# Autodesk Inventor assembly: Assembled Water Sensor Chassi
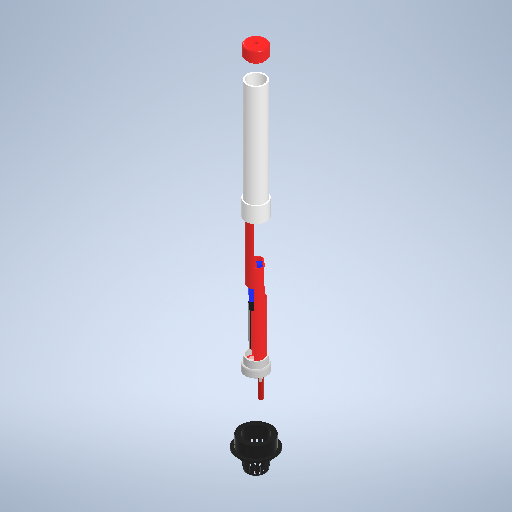
[picture p0: Inventor's stored thumbnail of the model, 512x512]
Saved by Autodesk Inventor 2025 (Build 290162000, 162)
## iProperties
Created: 2024-06-24
Part Number: Assembled Water Sensor Chassi
Document SubType Name: Assembly
Designer: track
Author: track
## Documents named in this file (14)
- C:\Users\track\OneDrive\Documents\In-Situ-Water-Quality-Sensor\System_development\Jocassee\V0.4.7\Water Sensor Chassi CAD\Assembled Water Sensor Chassi.iam
- C:\Users\track\OneDrive\Documents\In-Situ-Water-Quality-Sensor\System_development\Jocassee\V0.4.7\Water Sensor Chassi CAD\Water_Sensor_Cap.ipt
- C:\Users\track\OneDrive\Documents\In-Situ-Water-Quality-Sensor\System_development\Jocassee\V0.4.7\Tray_CAD_File\PCB tray CAD.ipt
- C:\Users\track\OneDrive\Documents\In-Situ-Water-Quality-Sensor\System_development\Jocassee\V0.4.7\Water Sensor Chassi CAD\Water Sensor Shaft (For assembly only).ipt
- C:\Users\track\OneDrive\Documents\In-Situ-Water-Quality-Sensor\System_development\Jocassee\V0.4.7\Water Sensor Chassi CAD\Male Adaptor to Water Sensor.ipt
- C:\Users\track\OneDrive\Documents\In-Situ-Water-Quality-Sensor\System_development\Jocassee\V0.4.7\Water Sensor Chassi CAD\Water Sensor Grate.ipt
- C:\Users\track\OneDrive\Documents\In-Situ-Water-Quality-Sensor\System_development\Jocassee\V0.4.7\Water Sensor Chassi CAD\Arc Water Sensor.ipt
- C:\Users\track\OneDrive\Documents\In-Situ-Water-Quality-Sensor\System_development\Jocassee\V0.4.7\Water Sensor Chassi CAD\Light Water Sensor.ipt
- C:\Users\track\OneDrive\Documents\In-Situ-Water-Quality-Sensor\System_development\Jocassee\V0.4.7\Water Sensor Chassi CAD\pH Sensor.ipt
- C:\Users\track\OneDrive\Documents\In-Situ-Water-Quality-Sensor\System_development\Jocassee\V0.4.7\Water Sensor Chassi CAD\Temp Water Sensor.ipt
- C:\Users\track\OneDrive\Documents\In-Situ-Water-Quality-Sensor\System_development\Jocassee\V0.4.7\Water Sensor Chassi CAD\PCB Board.ipt
- C:\Users\track\OneDrive\Documents\In-Situ-Water-Quality-Sensor\System_development\Jocassee\V0.4.7\Water Sensor Chassi CAD\Battery for Water Sensor.ipt
- C:\Users\track\OneDrive\Documents\In-Situ-Water-Quality-Sensor\System_development\Jocassee\V0.4.7\Tray_CAD_File\PCB Tray Top.ipt
- C:\Users\track\OneDrive\Documents\In-Situ-Water-Quality-Sensor\System_development\Jocassee\V0.4.7\Tray_CAD_File\PCB Battery Tray.ipt
## Components (13 placed, 13 different names)
1. PCB tray CAD:1 — Flush:2, Mate:2, Flush:3, Mate:3, Mate:4, Mate:5, Rigid:1, Mate:6, Mate:7, Flush:5, Mate:10, Mate:11, Mate:12, Mate:18, Mate:19, Mate:20, Mate:21, Mate:22
2. Water Sensor Shaft (For assembly only):1 — Mate:14, Mate:15
3. Water_Sensor_Cap:1 — Mate:15
4. Male Adaptor to Water Sensor:1 — Mate:11, Mate:12, Mate:13, Mate:14
5. Water Sensor Grate:1 — Mate:13
6. Arc Water Sensor:1 — Flush:5, Mate:10
7. Light Water Sensor:1 — Flush:3, Rigid:1
8. pH Sensor:1 — Mate:6, Mate:7
9. Temp Water Sensor:1 — Flush:2, Mate:2
10. PCB Board:1 — Mate:3, Mate:4, Mate:5
11. Battery for Water Sensor:1 — Mate:16, Flush:6, Mate:17
12. PCB Tray Top:1 — Mate:21, Mate:22
13. PCB Battery Tray:1 — Mate:16, Flush:6, Mate:17, Mate:18, Mate:19, Mate:20
## Relationships (24: Mate 19, Flush 4, WeldJoint 1)
- Flush:2: PCB tray CAD:1 ↔ Temp Water Sensor:1
- Mate:2: PCB tray CAD:1 ↔ Temp Water Sensor:1
- Flush:3: PCB tray CAD:1 ↔ Light Water Sensor:1
- Mate:3: PCB tray CAD:1 ↔ PCB Board:1
- Mate:4: PCB tray CAD:1 ↔ PCB Board:1
- Mate:5: PCB tray CAD:1 ↔ PCB Board:1
- Rigid:1 [WeldJoint]: PCB tray CAD:1 ↔ Light Water Sensor:1
- Mate:6: PCB tray CAD:1 ↔ pH Sensor:1
- Mate:7: PCB tray CAD:1 ↔ pH Sensor:1
- Flush:5: PCB tray CAD:1 ↔ Arc Water Sensor:1
- Mate:10: PCB tray CAD:1 ↔ Arc Water Sensor:1
- Mate:11: PCB tray CAD:1 ↔ Male Adaptor to Water Sensor:1
- Mate:12: PCB tray CAD:1 ↔ Male Adaptor to Water Sensor:1
- Mate:13: Male Adaptor to Water Sensor:1 ↔ Water Sensor Grate:1
- Mate:14: Water Sensor Shaft (For assembly only):1 ↔ Male Adaptor to Water Sensor:1
- Mate:15: Water Sensor Shaft (For assembly only):1 ↔ Water_Sensor_Cap:1
- Mate:16: Battery for Water Sensor:1 ↔ PCB Battery Tray:1
- Flush:6: Battery for Water Sensor:1 ↔ PCB Battery Tray:1
- Mate:17: Battery for Water Sensor:1 ↔ PCB Battery Tray:1
- Mate:18: PCB tray CAD:1 ↔ PCB Battery Tray:1
- Mate:19: PCB tray CAD:1 ↔ PCB Battery Tray:1
- Mate:20: PCB tray CAD:1 ↔ PCB Battery Tray:1
- Mate:21: PCB tray CAD:1 ↔ PCB Tray Top:1
- Mate:22: PCB tray CAD:1 ↔ PCB Tray Top:1
